# Autodesk Inventor assembly: Universal Shaft Angle
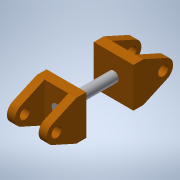
[picture p0: Inventor's stored thumbnail of the model, 180x180]
Saved by Autodesk Inventor 2022 (Build 260148000, 148)
## iProperties
Created: 2014-03-11
Part Number: Universal Shaft Angle
Document SubType Name: Assembly
Designer: John
Author: John
## Documents named in this file (3)
- C:\Users\helfenj\Desktop\Ex_Files_Autodesk_Inventor_2022_Essential_Training\Exercise Files\12_Using constraints to position parts\12_02\Universal Shaft Angle.iam
- C:\Users\helfenj\Desktop\Ex_Files_Autodesk_Inventor_2022_Essential_Training\Exercise Files\12_Using constraints to position parts\12_02\Joint.ipt
- C:\Users\helfenj\Desktop\Ex_Files_Autodesk_Inventor_2022_Essential_Training\Exercise Files\12_Using constraints to position parts\12_02\Connecting Rod.ipt
## Components (3 placed, 2 different names)
1. Joint:3 — Flush:1, Mate:1
2. Connecting Rod:1 — Flush:1, Mate:1, Flush:2, Mate:2
3. Joint:4 — Flush:2, Mate:2
## Relationships (4: Flush 2, Mate 2)
- Flush:1: Joint:3 ↔ Connecting Rod:1
- Mate:1: Joint:3 ↔ Connecting Rod:1
- Flush:2: Connecting Rod:1 ↔ Joint:4
- Mate:2: Connecting Rod:1 ↔ Joint:4
